# Autodesk Inventor assembly: Top_Assy
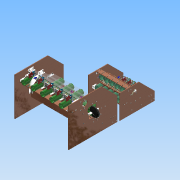
[picture p0: Inventor's stored thumbnail of the model, 180x180]
Saved by Autodesk Inventor 2018.1 (Build 221171000, 171)
## iProperties
Created: 2019-03-18
Part Number: Top_Assy
Document SubType Name: Assembly
Designer: James
Author: James
## Documents named in this file (3)
- C:\Users\admin\Desktop\Ball-Machine\Top Level\Top_Assy.iam
- C:\Users\admin\Desktop\Ball-Machine\Selection Sort\Selection_Assy.iam
- C:\Users\admin\Desktop\Ball-Machine\Pancake Sort\Pancake_Assy.iam
## Components (2 placed, 2 different names)
1. Selection_Assy:1 [sub-assembly] — Flush:1, Flush:2, Flush:3, Flush:4
2. Pancake_Assy:1 [sub-assembly] — Flush:4
## Relationships (4: Flush 4)
- Flush:1: Selection_Assy:1
- Flush:2: Selection_Assy:1
- Flush:3: Selection_Assy:1
- Flush:4 (110 mm): Selection_Assy:1 ↔ Pancake_Assy:1
